# Autodesk Inventor assembly: Functioning swerve drive (adjacent shaft axel)
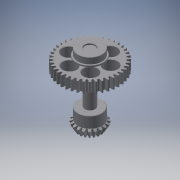
[picture p0: Inventor's stored thumbnail of the model, 180x180]
Saved by Autodesk Inventor 2019 (Build 230136000, 136)
## iProperties
Created: 2019-01-14
Part Number: Functioning swerve drive (adjacent shaft axel)
Document SubType Name: Assembly
Designer: josh
Author: josh
## Documents named in this file (6)
- D:\Synthesis Robots\Epsilon\Functioning swerve drive (adjacent shaft axel).iam
- D:\Synthesis Robots\Epsilon\20t 1-25mod bevel gear.ipt
- D:\Synthesis Robots\Epsilon\Bevel Input Shaft.ipt
- D:\Synthesis Robots\Epsilon\FR6ZZ Bearing_smart.ipt
- D:\Synthesis Robots\Epsilon\40T 20dp 375h_Inch - Spur gear 20DP 40T 14.5PA .372FW ---S40N3.0H2.0L0.25N.ipt
- D:\Synthesis Robots\Epsilon\500 Washer am-1001.ipt
## Components (7 placed, 5 different names)
1. 20t 1-25mod bevel gear:1
2. Bevel Input Shaft:1
3. FR6ZZ Bearing_smart:1
4. 40T 20dp 375h_Inch - Spur gear 20DP 40T 14.5PA .372FW ---S40N3.0H2.0L0.25N:1
5. 500 Washer am-1001:1
6. 500 Washer am-1001:2
7. FR6ZZ Bearing_smart:2
## Relationships (13: Mate 10, Flush 2, RevoluteJoint 1)
- [Mate]: Bevel Input Shaft:1 ↔ FR6ZZ Bearing_smart:1
- [Mate]: Bevel Input Shaft:1 ↔ 500 Washer am-1001:1
- [Mate]: Bevel Input Shaft:1 ↔ 40T 20dp 375h_Inch - Spur gear 20DP 40T 14.5PA .372FW ---S40N3.0H2.0L0.25N:1
- [Mate]: Bevel Input Shaft:1 ↔ 40T 20dp 375h_Inch - Spur gear 20DP 40T 14.5PA .372FW ---S40N3.0H2.0L0.25N:1
- [Flush]: Bevel Input Shaft:1 ↔ 40T 20dp 375h_Inch - Spur gear 20DP 40T 14.5PA .372FW ---S40N3.0H2.0L0.25N:1
- [Mate]: Bevel Input Shaft:1 ↔ 500 Washer am-1001:2
- [Mate]: Bevel Input Shaft:1 ↔ FR6ZZ Bearing_smart:2
- [Mate]: 500 Washer am-1001:2 ↔ FR6ZZ Bearing_smart:2
- [Mate]: Bevel Input Shaft:1 ↔ 500 Washer am-1001:2
- [Flush]: Bevel Input Shaft:1 ↔ 500 Washer am-1001:1
- [RevoluteJoint]: 20t 1-25mod bevel gear:1 ↔ Bevel Input Shaft:1
- [Mate]: FR6ZZ Bearing_smart:1 ↔ 500 Washer am-1001:1
- [Mate]: 20t 1-25mod bevel gear:1 ↔ Bevel Input Shaft:1
## Named parameters: d397_d206 = 0 mm, d196_d95_d168 = 0 mm, d205_d96_d169 = 0 mm, d208_d172 = 0 mm, d250_d173 = 0 mm, d251_d179 = 0 mm, d252_d184 = 0 mm, d260_d185 = 0 mm, d261_d186 = 0 mm, d265_d187 = 0 mm, d269_d190 = 0 mm, d283_d194 = 0 mm, d284_d195 = -120 deg, d346_d777 = 0 mm
